# Autodesk Inventor assembly: Roller Piston 4 Mount
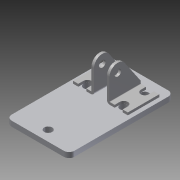
[picture p0: Inventor's stored thumbnail of the model, 180x180]
Saved by Autodesk Inventor 2014 (Build 180170000, 170)
## iProperties
Created: 2014-02-21
Part Number: Roller Piston 4 Mount
Document SubType Name: Assembly
Designer: Michael
Author: Michael
## Documents named in this file (3)
- C:\Users\Michael\Documents\GitHub\2014buildCAD\Duluth Collector\Roller Piston 4 Mount.iam
- C:\Users\Michael\Documents\GitHub\2014buildCAD\Duluth Collector\Foot Bracket Mount (McMaster Part #6498K710).ipt
- C:\Users\Michael\Documents\GitHub\2014buildCAD\Duluth Collector\Roller Pneumatic Back Connector (Custom).ipt
## Components (2 placed, 2 different names)
1. Foot Bracket Mount (McMaster Part #6498K710):1 — Mate:1, Mate:2, Mate:3
2. Roller Pneumatic Back Connector (Custom):1 — Mate:1, Mate:2, Mate:3
## Relationships (3: Mate 3)
- Mate:1: Foot Bracket Mount (McMaster Part #6498K710):1 ↔ Roller Pneumatic Back Connector (Custom):1
- Mate:2: Foot Bracket Mount (McMaster Part #6498K710):1 ↔ Roller Pneumatic Back Connector (Custom):1
- Mate:3: Foot Bracket Mount (McMaster Part #6498K710):1 ↔ Roller Pneumatic Back Connector (Custom):1
